# Autodesk Inventor assembly: v2RevA
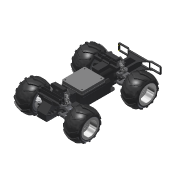
[picture p0: Inventor's stored thumbnail of the model, 180x180]
Saved by Autodesk Inventor 2015 (Build 190159000, 159)
## iProperties
Created: 2013-12-30
Part Number: v2RevA
Document SubType Name: Assembly
Designer: davidgitz
Author: davidgitz
## Documents named in this file (18)
- C:\SharedDrive\Dropbox\FAST Robotics\Products\FAST_ROVER\810002_ASY-FAST ROVER v2\813004_FAST ROVER v2 CHASSIS\813005_Hummer H2 Chassis\813005_Hummer H2 Chassis.iam
- C:\SharedDrive\Dropbox\FAST Robotics\Products\FAST_ROVER\810002_ASY-FAST ROVER v2\813004_FAST ROVER v2 CHASSIS\813005_Hummer H2 Chassis\Drive Axle.ipt
- C:\SharedDrive\Dropbox\FAST Robotics\Products\FAST_ROVER\810002_ASY-FAST ROVER v2\813004_FAST ROVER v2 CHASSIS\813005_Hummer H2 Chassis\Rear Axle Housing.ipt
- C:\SharedDrive\Dropbox\FAST Robotics\Products\FAST_ROVER\810002_ASY-FAST ROVER v2\813004_FAST ROVER v2 CHASSIS\813005_Hummer H2 Chassis\Elec Cover.ipt
- C:\SharedDrive\Dropbox\FAST Robotics\Products\FAST_ROVER\810002_ASY-FAST ROVER v2\813004_FAST ROVER v2 CHASSIS\813005_Hummer H2 Chassis\Shock Plate - Top (Left).ipt
- C:\SharedDrive\Dropbox\FAST Robotics\Products\FAST_ROVER\810002_ASY-FAST ROVER v2\813004_FAST ROVER v2 CHASSIS\813005_Hummer H2 Chassis\Shock Plate - Bottom (Left).ipt
- C:\SharedDrive\Dropbox\FAST Robotics\Products\FAST_ROVER\810002_ASY-FAST ROVER v2\813004_FAST ROVER v2 CHASSIS\813005_Hummer H2 Chassis\Shock Plate - Bottom (Right).ipt
- C:\SharedDrive\Dropbox\FAST Robotics\Products\FAST_ROVER\810002_ASY-FAST ROVER v2\813004_FAST ROVER v2 CHASSIS\813005_Hummer H2 Chassis\Shock Plate - Top (Right).ipt
- C:\SharedDrive\Dropbox\FAST Robotics\Products\FAST_ROVER\810002_ASY-FAST ROVER v2\813004_FAST ROVER v2 CHASSIS\813005_Hummer H2 Chassis\Shock Mount - Top.ipt
- C:\SharedDrive\Dropbox\FAST Robotics\Products\FAST_ROVER\810002_ASY-FAST ROVER v2\813004_FAST ROVER v2 CHASSIS\813005_Hummer H2 Chassis\FrontHousing.ipt
- C:\SharedDrive\Dropbox\FAST Robotics\Products\FAST_ROVER\810002_ASY-FAST ROVER v2\813004_FAST ROVER v2 CHASSIS\813005_Hummer H2 Chassis\RearHousing.ipt
- C:\SharedDrive\Dropbox\FAST Robotics\Products\FAST_ROVER\810002_ASY-FAST ROVER v2\813004_FAST ROVER v2 CHASSIS\813005_Hummer H2 Chassis\LargeLeftWheel.ipt
- C:\SharedDrive\Dropbox\FAST Robotics\Products\FAST_ROVER\810002_ASY-FAST ROVER v2\813004_FAST ROVER v2 CHASSIS\813005_Hummer H2 Chassis\LargeRightWheel.ipt
- C:\SharedDrive\Dropbox\FAST Robotics\Products\FAST_ROVER\810002_ASY-FAST ROVER v2\813004_FAST ROVER v2 CHASSIS\813005_Hummer H2 Chassis\Front Axle Housing.ipt
- C:\SharedDrive\Dropbox\FAST Robotics\Products\FAST_ROVER\810002_ASY-FAST ROVER v2\813004_FAST ROVER v2 CHASSIS\813005_Hummer H2 Chassis\Front Axle Body.ipt
- C:\SharedDrive\Dropbox\FAST Robotics\Products\FAST_ROVER\810002_ASY-FAST ROVER v2\813004_FAST ROVER v2 CHASSIS\813005_Hummer H2 Chassis\BackBumper.ipt
- C:\SharedDrive\Dropbox\FAST Robotics\Products\FAST_ROVER\810002_ASY-FAST ROVER v2\813004_FAST ROVER v2 CHASSIS\813005_Hummer H2 Chassis\Shock Mount - Bottom.ipt
- C:\SharedDrive\Dropbox\FAST Robotics\Products\FAST_ROVER\810002_ASY-FAST ROVER v2\813004_FAST ROVER v2 CHASSIS\813005_Hummer H2 Chassis\Shock Spring.ipt
## Components (38 placed, 22 different names)
1. Drive Axle:1 — Mate:9, Insert:2, Insert:36
2. Drive Axle:2 — Mate:7, Insert:1, Insert:35
3. Drive Axle:3 — Mate:13, Insert:6, Insert:25
4. Drive Axle:4 — Mate:11, Insert:5, Insert:26
5. Elec Cover:1 — Flush:43, Mate:67, Mate:68
6. FrontLeft_Wheel — Mate:7, Insert:1
7. FrontRight_Wheel — Mate:9, Insert:2
8. BackLeft_Wheel — Mate:13, Insert:6
9. BackRight_Wheel — Mate:11, Insert:5
10. Shock Plate - Top (Left):1 — Insert:17, Insert:21, Insert:38
11. Shock Plate - Bottom (Left):1 — Insert:18, Insert:22
12. Shock Plate - Bottom (Right):1 — Insert:20, Insert:23
13. Shock Plate - Top (Right):1 — Insert:19, Insert:24, Insert:40
14. FrontHousing:1 — Insert:13, Insert:15, Angle:4, Flush:16, Insert:27, Insert:28, Mate:22, Flush:17, Mate:23, Mate:25, Mate:29, Mate:31, Flush:31
15. Shock Plate - Bottom (Left):2 — Insert:27, Insert:30
16. Shock Plate - Top (Left):2 — Insert:13, Insert:29, Insert:37
17. Shock Plate - Bottom (Right):2 — Insert:28, Insert:32
18. Shock Plate - Top (Right):2 — Insert:15, Insert:31, Insert:39
19. RearHousing:1 — Insert:17, Insert:18, Insert:19, Insert:20, Mate:22, Flush:17, Mate:23, Mate:24, Flush:20, Mate:27, Mate:34, Mate:35, Mate:67, Mate:68
20. Rear Axle Housing:3 — Insert:21, Insert:22, Insert:25
21. Rear Axle Housing:4 — Insert:23, Insert:24, Insert:26
22. Front Left Axle Housing:1 — Insert:29, Insert:30, Insert:33, DRIVEN-FL WHEEL ANGLE
23. Front Right Axle Housing:2 — Insert:31, Insert:32, Insert:34, DRIVEN-FR WHEEL ANGLE
24. Front Left Axle Body:1 — Insert:33, Insert:35, DRIVEN-FL WHEEL ANGLE
25. Front Right Axle Body:2 — Insert:34, Insert:36, DRIVEN-FR WHEEL ANGLE
26. BackBumper:1 — Flush:20, Mate:27, Flush:21
27. Shock Mount - Bottom:1 — Insert:40, Mate:33, Mate:52
28. Shock Mount - Top:2 — Mate:33, Mate:34, Mate:50, Mate:51
29. Shock Mount - Bottom:2 — Insert:39, Mate:30, Mate:46
30. Shock Mount - Top:3 — Mate:30, Mate:31, Mate:44, Mate:45
31. Shock Mount - Bottom:3 — Insert:37, Mate:28, Mate:41, DRIVEN-SHOCK HEIGHT
32. Shock Mount - Top:4 — Mate:32, Mate:35, Mate:47, Mate:48
33. Shock Mount - Bottom:4 — Insert:38, Mate:32, Mate:49
34. FL Shock Mount — Mate:28, Mate:29, Mate:40, Mate:42, DRIVEN-SHOCK HEIGHT
35. Shock Spring:1 — Mate:40, Mate:41, Mate:42
36. Shock Spring:2 — Mate:44, Mate:45, Mate:46
37. Shock Spring:3 — Mate:47, Mate:48, Mate:49
38. Shock Spring:4 — Mate:50, Mate:51, Mate:52
## Relationships (73: Mate 32, Insert 30, Flush 8, Angle 3)
- Flush:5
- Mate:7: Drive Axle:2 ↔ FrontLeft_Wheel
- Insert:1: Drive Axle:2 ↔ FrontLeft_Wheel
- Mate:9: Drive Axle:1 ↔ FrontRight_Wheel
- Insert:2: Drive Axle:1 ↔ FrontRight_Wheel
- Mate:11: Drive Axle:4 ↔ BackRight_Wheel
- Insert:5: Drive Axle:4 ↔ BackRight_Wheel
- Mate:13: Drive Axle:3 ↔ BackLeft_Wheel
- Insert:6: Drive Axle:3 ↔ BackLeft_Wheel
- Insert:13: FrontHousing:1 ↔ Shock Plate - Top (Left):2
- Insert:15: FrontHousing:1 ↔ Shock Plate - Top (Right):2
- Insert:17: Shock Plate - Top (Left):1 ↔ RearHousing:1
- Insert:18: Shock Plate - Bottom (Left):1 ↔ RearHousing:1
- Insert:19: Shock Plate - Top (Right):1 ↔ RearHousing:1
- Insert:20: Shock Plate - Bottom (Right):1 ↔ RearHousing:1
- Insert:21: Shock Plate - Top (Left):1 ↔ Rear Axle Housing:3
- Insert:22: Shock Plate - Bottom (Left):1 ↔ Rear Axle Housing:3
- Insert:23: Shock Plate - Bottom (Right):1 ↔ Rear Axle Housing:4
- Insert:24: Shock Plate - Top (Right):1 ↔ Rear Axle Housing:4
- Insert:25: Drive Axle:3 ↔ Rear Axle Housing:3
- Insert:26: Drive Axle:4 ↔ Rear Axle Housing:4
- Angle:4 (0 deg): FrontHousing:1
- Flush:16: FrontHousing:1
- Insert:27: FrontHousing:1 ↔ Shock Plate - Bottom (Left):2
- Insert:28: FrontHousing:1 ↔ Shock Plate - Bottom (Right):2
- Insert:29: Shock Plate - Top (Left):2 ↔ Front Left Axle Housing:1
- Insert:30: Shock Plate - Bottom (Left):2 ↔ Front Left Axle Housing:1
- Insert:31: Shock Plate - Top (Right):2 ↔ Front Right Axle Housing:2
- Insert:32: Shock Plate - Bottom (Right):2 ↔ Front Right Axle Housing:2
- Insert:33 (0.6604 mm): Front Left Axle Housing:1 ↔ Front Left Axle Body:1
- Insert:34 (0.6604 mm): Front Right Axle Housing:2 ↔ Front Right Axle Body:2
- Insert:35: Drive Axle:2 ↔ Front Left Axle Body:1
- Insert:36: Drive Axle:1 ↔ Front Right Axle Body:2
- Mate:22: FrontHousing:1 ↔ RearHousing:1
- Flush:17: FrontHousing:1 ↔ RearHousing:1
- Mate:23: FrontHousing:1 ↔ RearHousing:1
- Mate:24: RearHousing:1
- Mate:25: FrontHousing:1
- Flush:20: RearHousing:1 ↔ BackBumper:1
- Mate:27: RearHousing:1 ↔ BackBumper:1
- Flush:21: BackBumper:1
- Insert:37 (0.889 mm): Shock Plate - Top (Left):2 ↔ Shock Mount - Bottom:3
- Insert:38 (0.889 mm): Shock Plate - Top (Left):1 ↔ Shock Mount - Bottom:4
- Insert:39 (0.889 mm): Shock Plate - Top (Right):2 ↔ Shock Mount - Bottom:2
- Insert:40 (0.889 mm): Shock Plate - Top (Right):1 ↔ Shock Mount - Bottom:1
- Mate:28: Shock Mount - Bottom:3 ↔ FL Shock Mount
- Mate:29: FrontHousing:1 ↔ FL Shock Mount
- Mate:30: Shock Mount - Bottom:2 ↔ Shock Mount - Top:3
- Mate:31: FrontHousing:1 ↔ Shock Mount - Top:3
- Mate:32: Shock Mount - Top:4 ↔ Shock Mount - Bottom:4
- Mate:33: Shock Mount - Bottom:1 ↔ Shock Mount - Top:2
- Mate:34: RearHousing:1 ↔ Shock Mount - Top:2
- Mate:35: RearHousing:1 ↔ Shock Mount - Top:4
- Flush:29
- DRIVEN-FL WHEEL ANGLE [Angle] (0 deg): Front Left Axle Housing:1 ↔ Front Left Axle Body:1
- DRIVEN-FR WHEEL ANGLE [Angle] (0 deg): Front Right Axle Housing:2 ↔ Front Right Axle Body:2
- Mate:40: FL Shock Mount ↔ Shock Spring:1
- Mate:41: Shock Mount - Bottom:3 ↔ Shock Spring:1
- Mate:42: FL Shock Mount ↔ Shock Spring:1
- DRIVEN-SHOCK HEIGHT [Mate] (38.1 mm): Shock Mount - Bottom:3 ↔ FL Shock Mount
- Mate:44: Shock Mount - Top:3 ↔ Shock Spring:2
- Mate:45: Shock Mount - Top:3 ↔ Shock Spring:2
- Mate:46: Shock Mount - Bottom:2 ↔ Shock Spring:2
- Mate:47: Shock Mount - Top:4 ↔ Shock Spring:3
- Mate:48: Shock Mount - Top:4 ↔ Shock Spring:3
- Mate:49: Shock Mount - Bottom:4 ↔ Shock Spring:3
- Mate:50: Shock Mount - Top:2 ↔ Shock Spring:4
- Mate:51: Shock Mount - Top:2 ↔ Shock Spring:4
- Mate:52: Shock Mount - Bottom:1 ↔ Shock Spring:4
- Flush:31 (-13.97 mm): FrontHousing:1
- Flush:43: Elec Cover:1
- Mate:67: Elec Cover:1 ↔ RearHousing:1
- Mate:68: Elec Cover:1 ↔ RearHousing:1
